# Autodesk Inventor assembly: RS-381_MIR1
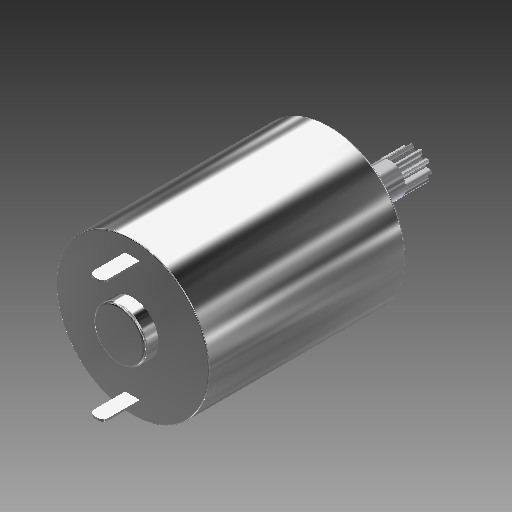
[picture p0: Inventor's stored thumbnail of the model, 512x512]
Saved by Autodesk Inventor 2019.2 (Build 232265000, 265)
## iProperties
Part Number: RS-381_MIR1
Material: 一般
Document SubType Name: Assembly
Designer: 雪村
Mass: 85 g
Surface Area: 56.1079 cm^2
Volume: 26.0295 cm^3
Density: 3.26552 g/cm^3
Author: 雪村
## Documents named in this file (3)
- C:\Users\white\Documents\SRDC\SRDC\Inventor_2017\2018年機体\パーツ\RS-381_MIR1.iam
- C:\Users\white\Documents\SRDC\SRDC\Inventor_2017\2018年機体\パーツ\RS-381_MIR1.ipt
- C:\Users\white\Documents\SRDC\SRDC\Inventor_2017\2018年機体\パーツ\ピニオン11_MIR1.ipt
## Components (2 placed, 2 different names)
1. RS-381_MIR1:1 — 挿入:1
2. ピニオン11_MIR1:1 — 挿入:1
## Relationships (1: Insert 1)
- 挿入:1 [Insert]: RS-381_MIR1:1 ↔ ピニオン11_MIR1:1
